# Autodesk Inventor assembly: TH1-001_CAM1
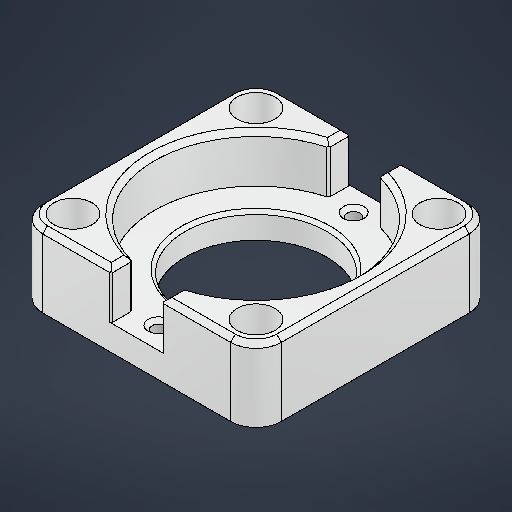
[picture p0: Inventor's stored thumbnail of the model, 512x512]
Saved by Autodesk Inventor 2025.3 (Build 293356000, 356)
## iProperties
Created: 2024-11-12
Part Number: TH1-001_CAM1
Document SubType Name: Assembly
Designer: fablabadmin
Author: fablabadmin
## Documents named in this file (8)
- C:\Users\fablabadmin\Documents\_Benjamin_S\_3dCAD\_WEDU\ToolHolder1\_TH1-001_CAM\TH1-001_CAM1.iam
- C:\Users\fablabadmin\Documents\_Benjamin_S\_3dCAD\_Config\KemmlerVise\OP1-KemmlerVise.iam
- C:\Users\fablabadmin\Documents\_Benjamin_S\_3dCAD\_Config\KemmlerVise\OP2-KemmlerVise.iam
- C:\Users\fablabadmin\Documents\Inventor\Content Center Files\R2024\en-US\StandardJaw\JawSTD-Aluminum 6061.ipt
- C:\Users\fablabadmin\Documents\_Benjamin_S\_3dCAD\_WEDU\ToolHolder1\TH1-001.ipt
- C:\Users\fablabadmin\Documents\_Benjamin_S\_3dCAD\_WEDU\ToolHolder1\_TH1-001_CAM\OP1Stock.ipt
- C:\Users\fablabadmin\Documents\Inventor\Content Center Files\R2024\en-US\EndStop\EndStop-Generic.ipt
- C:\Users\fablabadmin\Documents\_Benjamin_S\_3dCAD\_Config\_CAM_SIM\FixtureParts\parallels3mm.xlsx
## Components (9 placed, 6 different names)
1. TH1-001:1 — Flush:7, Mate:10, Mate:11, Mate:12, Mate:14, Mate:19
2. OP1Stock:1 — Flush:5, Flush:6, Flush:7, Mate:7, Mate:8, Mate:9
3. EndStop EndStop-Generic:1 — Mate:17, Mate:18, Mate:19
4. OP1-KemmlerVise:1 [sub-assembly] — Mate:1, Mate:2, Flush:1, Mate:3, Mate:9, Flush:8
5. JawStandard JawSTD-Aluminum 6061:1 — Mate:1, Flush:1, Flush:2, Mate:3, Mate:7
6. JawStandard JawSTD-Aluminum 6061:2 — Mate:2, Flush:2, Mate:8
7. OP2-KemmlerVise:1 [sub-assembly] — Mate:4, Mate:5, Flush:3, Mate:6, Mate:12, Mate:13, Mate:15
8. JawStandard JawSTD-Aluminum 6061:3 — Mate:4, Flush:3, Flush:4, Mate:6, Mate:10, Mate:17, Mate:18
9. JawStandard JawSTD-Aluminum 6061:4 — Mate:5, Flush:4, Mate:11
## Relationships (27: Mate 19, Flush 8)
- Mate:1: OP1-KemmlerVise:1 ↔ JawStandard JawSTD-Aluminum 6061:1
- Mate:2: OP1-KemmlerVise:1 ↔ JawStandard JawSTD-Aluminum 6061:2
- Flush:1: OP1-KemmlerVise:1 ↔ JawStandard JawSTD-Aluminum 6061:1
- Flush:2: JawStandard JawSTD-Aluminum 6061:1 ↔ JawStandard JawSTD-Aluminum 6061:2
- Mate:3: OP1-KemmlerVise:1 ↔ JawStandard JawSTD-Aluminum 6061:1
- Mate:4: OP2-KemmlerVise:1 ↔ JawStandard JawSTD-Aluminum 6061:3
- Mate:5: OP2-KemmlerVise:1 ↔ JawStandard JawSTD-Aluminum 6061:4
- Flush:3: OP2-KemmlerVise:1 ↔ JawStandard JawSTD-Aluminum 6061:3
- Flush:4: JawStandard JawSTD-Aluminum 6061:3 ↔ JawStandard JawSTD-Aluminum 6061:4
- Mate:6: OP2-KemmlerVise:1 ↔ JawStandard JawSTD-Aluminum 6061:3
- Flush:5: OP1Stock:1
- Flush:6: OP1Stock:1
- Flush:7 (-0.5 mm): TH1-001:1 ↔ OP1Stock:1
- Mate:7: OP1Stock:1 ↔ JawStandard JawSTD-Aluminum 6061:1
- Mate:8: OP1Stock:1 ↔ JawStandard JawSTD-Aluminum 6061:2
- Mate:9 (41 mm): OP1Stock:1 ↔ OP1-KemmlerVise:1
- Flush:8: OP1-KemmlerVise:1
- Mate:10: TH1-001:1 ↔ JawStandard JawSTD-Aluminum 6061:3
- Mate:11: TH1-001:1 ↔ JawStandard JawSTD-Aluminum 6061:4
- Mate:12 (28 mm): TH1-001:1 ↔ OP2-KemmlerVise:1
- Mate:13: OP2-KemmlerVise:1
- Mate:14: TH1-001:1
- Mate:15: OP2-KemmlerVise:1
- Mate:16
- Mate:17: EndStop EndStop-Generic:1 ↔ JawStandard JawSTD-Aluminum 6061:3
- Mate:18: EndStop EndStop-Generic:1 ↔ JawStandard JawSTD-Aluminum 6061:3
- Mate:19: TH1-001:1 ↔ EndStop EndStop-Generic:1
## Named parameters: PRL13 = 13 mm, PRL16 = 16 mm, PRL19 = 19 mm, PRL22 = 22 mm, PRL28 = 28 mm, PRL31 = 31 mm, PRL35 = 35 mm, PRL38 = 38 mm, PRL41 = 41 mm
